# Autodesk Inventor assembly: DriveTrainPlateMecanum2017-18BackUp
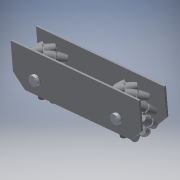
[picture p0: Inventor's stored thumbnail of the model, 180x180]
Saved by Autodesk Inventor 2017 (Build 210142000, 142)
## iProperties
Created: 2017-09-16
Part Number: DriveTrainPlateMecanum2017-18BackUp
Document SubType Name: Assembly
Designer: User
Author: User
## Documents named in this file (3)
- C:\Robotics\CAD\2016-17_CAD\Custom COTS\DriveTrainPlateMecanum2017-18BackUp.iam
- C:\Robotics\CAD\2017-18_CAD\MecanumDriveTrainPlate17-18.ipt
- C:\Robotics\CAD\2017-18_CAD\LeftDriveTrainMecanum2017-18.iam
## Components (4 placed, 2 different names)
1. MecanumDriveTrainPlate17-18:1 — Mate:1, Mate:2, Mate:3, Mate:4, Mate:8
2. LeftDriveTrainMecanum2017-18:1 [sub-assembly] — Mate:1, Mate:2, Mate:5, Mate:8, Mate:9
3. LeftDriveTrainMecanum2017-18:2 [sub-assembly] — Mate:3, Mate:4, Mate:6, Mate:7
4. MecanumDriveTrainPlate17-18:2 — Mate:5, Mate:6, Mate:7, Mate:9
## Relationships (9: Mate 9)
- Mate:1: MecanumDriveTrainPlate17-18:1 ↔ LeftDriveTrainMecanum2017-18:1
- Mate:2: MecanumDriveTrainPlate17-18:1 ↔ LeftDriveTrainMecanum2017-18:1
- Mate:3: MecanumDriveTrainPlate17-18:1 ↔ LeftDriveTrainMecanum2017-18:2
- Mate:4: MecanumDriveTrainPlate17-18:1 ↔ LeftDriveTrainMecanum2017-18:2
- Mate:5: LeftDriveTrainMecanum2017-18:1 ↔ MecanumDriveTrainPlate17-18:2
- Mate:6: LeftDriveTrainMecanum2017-18:2 ↔ MecanumDriveTrainPlate17-18:2
- Mate:7: LeftDriveTrainMecanum2017-18:2 ↔ MecanumDriveTrainPlate17-18:2
- Mate:8: MecanumDriveTrainPlate17-18:1 ↔ LeftDriveTrainMecanum2017-18:1
- Mate:9: LeftDriveTrainMecanum2017-18:1 ↔ MecanumDriveTrainPlate17-18:2
